# Autodesk Inventor assembly: NEMA 23 - 56mm
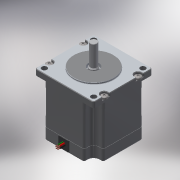
[picture p0: Inventor's stored thumbnail of the model, 180x180]
Saved by Autodesk Inventor 2020.3 (Build 243373000, 373)
## iProperties
Created: 2021-03-08
Part Number: NEMA 23 - 56mm
Description: STEP AP214
Document SubType Name: Assembly
Designer: justi
Sending System: SolidWorks 2020
Preprocessor: SwSTEP 2.0
Title: NEMA 23 - 56mm.STEP
Revision Number: ANY
## Documents named in this file (3)
- F:\UQ Engineering\2021 ~ 5th Year\Semester 2\METR4911-THESIS\FarmBot CAD\FarmBotV1\NEMA 23 - 56mm.iam
- F:\UQ Engineering\2021 ~ 5th Year\Semester 2\METR4911-THESIS\FarmBot CAD\FarmBotV1\NEMA 23 - 56mm.ipt
- F:\UQ Engineering\2021 ~ 5th Year\Semester 2\METR4911-THESIS\FarmBot CAD\FarmBotV1\pan head cross recess screw_iso_ISO 7045 - M3 x 10 - Z - 10N.ipt
## Components (5 placed, 5 different names)
1. NEMA 23 - 56mm_1 — Mate:1, Mate:2, Mate:3, Mate:4, Mate:5, Mate:6, Mate:7, Mate:8, Flush:1
2. pan head cross recess screw_iso_ISO 7045 - M3 x 10 - Z - 10N_2 — Mate:1, Mate:2
3. pan head cross recess screw_iso_ISO 7045 - M3 x 10 - Z - 10N_3 — Mate:3, Mate:4
4. pan head cross recess screw_iso_ISO 7045 - M3 x 10 - Z - 10N_4 — Mate:5, Mate:6
5. pan head cross recess screw_iso_ISO 7045 - M3 x 10 - Z - 10N_5 — Mate:7, Mate:8
## Relationships (9: Mate 8, Flush 1)
- Mate:1: NEMA 23 - 56mm_1 ↔ pan head cross recess screw_iso_ISO 7045 - M3 x 10 - Z - 10N_2
- Mate:2: NEMA 23 - 56mm_1 ↔ pan head cross recess screw_iso_ISO 7045 - M3 x 10 - Z - 10N_2
- Mate:3: NEMA 23 - 56mm_1 ↔ pan head cross recess screw_iso_ISO 7045 - M3 x 10 - Z - 10N_3
- Mate:4: NEMA 23 - 56mm_1 ↔ pan head cross recess screw_iso_ISO 7045 - M3 x 10 - Z - 10N_3
- Mate:5: NEMA 23 - 56mm_1 ↔ pan head cross recess screw_iso_ISO 7045 - M3 x 10 - Z - 10N_4
- Mate:6: NEMA 23 - 56mm_1 ↔ pan head cross recess screw_iso_ISO 7045 - M3 x 10 - Z - 10N_4
- Mate:7: NEMA 23 - 56mm_1 ↔ pan head cross recess screw_iso_ISO 7045 - M3 x 10 - Z - 10N_5
- Mate:8: NEMA 23 - 56mm_1 ↔ pan head cross recess screw_iso_ISO 7045 - M3 x 10 - Z - 10N_5
- Flush:1: NEMA 23 - 56mm_1
